# Autodesk Inventor assembly: tire
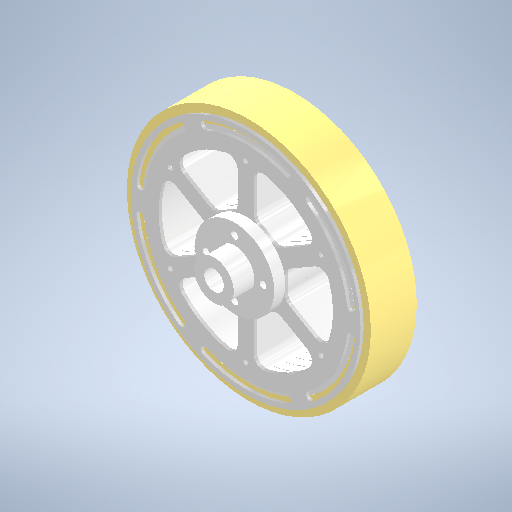
[picture p0: Inventor's stored thumbnail of the model, 512x512]
Saved by Autodesk Inventor 2025.1 (Build 291241000, 241)
## iProperties
Created: 2024-10-03
Part Number: tire
Document SubType Name: Assembly
Designer: yuki0520
Author: yuki0520
## Documents named in this file (5)
- C:\Users\yuki0520\OneDrive\ドキュメント\Inventor\2025_nhk\tanaka\nageru\pakuriz\tire.iam
- C:\Users\yuki0520\OneDrive\ドキュメント\Inventor\2025_nhk\tanaka\nageru\pakuriz\TH22_POM_roller_sn.ipt
- C:\Users\yuki0520\OneDrive\ドキュメント\Inventor\2025_nhk\tanaka\nageru\pakuriz\TH22_Urethane_roller_sn.ipt
- C:\Users\yuki0520\OneDrive\ドキュメント\Inventor\2025_nhk\tanaka\nageru\pakuriz\TH22_AlBoard_roller_sn.ipt
- C:\Users\yuki0520\OneDrive\ドキュメント\Inventor\2025_nhk\tanaka\nageru\pakuriz\TH22_3DP_roller_fixer_sn.ipt
## Components (9 placed, 4 different names)
1. TH22_POM_roller_sn:1 — 挿入:4, 挿入:6
2. TH22_POM_roller_sn:2 — 挿入:3, 正接:1, フラッシュ:1, 挿入:5
3. TH22_POM_roller_sn:3 — 挿入:2, 挿入:4
4. TH22_POM_roller_sn:4 — 挿入:1, 挿入:3
5. TH22_POM_roller_sn:5 — 挿入:1, 挿入:2
6. TH22_Urethane_roller_sn:1 — 正接:1, フラッシュ:1
7. TH22_AlBoard_roller_sn:1 — 挿入:6
8. TH22_AlBoard_roller_sn:2 — 挿入:5, 挿入:7, 挿入:8
9. TH22_3DP_roller_fixer_sn:1 — 挿入:7, 挿入:8
## Relationships (10: Insert 8, Tangent 1, Flush 1)
- 挿入:1 [Insert]: TH22_POM_roller_sn:4 ↔ TH22_POM_roller_sn:5
- 挿入:2 [Insert]: TH22_POM_roller_sn:3 ↔ TH22_POM_roller_sn:5
- 挿入:3 [Insert]: TH22_POM_roller_sn:2 ↔ TH22_POM_roller_sn:4
- 挿入:4 [Insert]: TH22_POM_roller_sn:1 ↔ TH22_POM_roller_sn:3
- 正接:1 [Tangent]: TH22_POM_roller_sn:2 ↔ TH22_Urethane_roller_sn:1
- フラッシュ:1 [Flush]: TH22_POM_roller_sn:2 ↔ TH22_Urethane_roller_sn:1
- 挿入:5 [Insert]: TH22_POM_roller_sn:2 ↔ TH22_AlBoard_roller_sn:2
- 挿入:6 [Insert]: TH22_POM_roller_sn:1 ↔ TH22_AlBoard_roller_sn:1
- 挿入:7 [Insert]: TH22_AlBoard_roller_sn:2 ↔ TH22_3DP_roller_fixer_sn:1
- 挿入:8 [Insert]: TH22_AlBoard_roller_sn:2 ↔ TH22_3DP_roller_fixer_sn:1
